# Autodesk Inventor assembly: canaletaDerecha
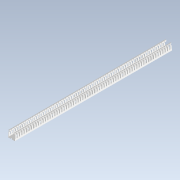
[picture p0: Inventor's stored thumbnail of the model, 180x180]
Saved by Autodesk Inventor 2021 (Build 250183000, 183)
## iProperties
Created: 2021-07-05
Part Number: canaletaDerecha
Document SubType Name: Assembly
Designer: Andrés Holguín
Author: Andrés Holguín
## Documents named in this file (2)
- C:\Users\andre\Documents\GitHub\Dis.-Mecatronico-E6\inventor proyecto\Tablero\Canaletas\canaletaDerecha.iam
- C:\Users\andre\Documents\GitHub\Dis.-Mecatronico-E6\inventor proyecto\Tablero\Canaletas\7308-1.iam
## Components (7 placed, 1 different names)
1. 7308-1:3 [sub-assembly] — Rigid:3, Mate:4, Angle:4
2. 7308-1:4 [sub-assembly] — Rigid:3, Rigid:4
3. 7308-1:5 [sub-assembly] — Rigid:4, Rigid:5
4. 7308-1:6 [sub-assembly] — Rigid:5, Mate:1, Angle:1, Rigid:8
5. 7308-1:7 [sub-assembly] — Rigid:6, Mate:2, Angle:2
6. 7308-1:8 [sub-assembly] — Rigid:6, Rigid:7
7. 7308-1:9 [sub-assembly] — Rigid:7, Rigid:8
## Relationships (12: WeldJoint 6, Mate 3, Angle 3)
- Rigid:3 [WeldJoint]: 7308-1:3 ↔ 7308-1:4
- Rigid:4 [WeldJoint]: 7308-1:4 ↔ 7308-1:5
- Rigid:5 [WeldJoint]: 7308-1:5 ↔ 7308-1:6
- Mate:1: 7308-1:6
- Angle:1 (45 deg): 7308-1:6
- Rigid:6 [WeldJoint]: 7308-1:7 ↔ 7308-1:8
- Rigid:7 [WeldJoint]: 7308-1:8 ↔ 7308-1:9
- Rigid:8 [WeldJoint]: 7308-1:6 ↔ 7308-1:9
- Mate:2: 7308-1:7
- Angle:2 (-45 deg): 7308-1:7
- Mate:4: 7308-1:3
- Angle:4 (45 deg): 7308-1:3
